# Autodesk Inventor assembly: GFRP_T2_01
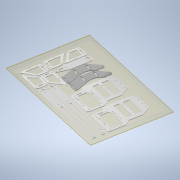
[picture p0: Inventor's stored thumbnail of the model, 180x180]
Saved by Autodesk Inventor 2020 (Build 240168000, 168)
## iProperties
Created: 2021-08-27
Part Number: GFRP_T2_01
Document SubType Name: Assembly
Designer: Masato
Author: Masato
## Documents named in this file (7)
- C:\Users\naoki\Documents\Inventor\CitBrains\git_clone\OpenPlatform167\CAMの確認用\OpenPlatform_ver3_0\cam\GFRP_T2_01.iam
- C:\Users\naoki\Documents\Inventor\CitBrains\git_clone\OpenPlatform167\CAMの確認用\OpenPlatform_ver3_0\cam\Disposable_Board.ipt
- C:\Users\naoki\Documents\Inventor\CitBrains\git_clone\OpenPlatform167\CAMの確認用\OpenPlatform_ver3_0\UpperBody\Head\Head_side_frame.ipt
- C:\Users\naoki\Documents\Inventor\CitBrains\git_clone\OpenPlatform167\CAMの確認用\OpenPlatform_ver3_0\UpperBody\Trunk\Trunk_upper_flank_frame.ipt
- C:\Users\naoki\Documents\Inventor\CitBrains\git_clone\OpenPlatform167\CAMの確認用\OpenPlatform_ver3_0\UpperBody\Arm\ForeArm_outside_frame.ipt
- C:\Users\naoki\Documents\Inventor\CitBrains\git_clone\OpenPlatform167\CAMの確認用\OpenPlatform_ver3_0\UpperBody\Arm\ForeArm_inside_frame.ipt
- C:\Users\naoki\Documents\Inventor\CitBrains\git_clone\OpenPlatform167\CAMの確認用\OpenPlatform_ver3_0\UpperBody\Arm\UpperArm_side_frame.ipt
## Components (13 placed, 6 different names)
1. Disposable_Board:1 — メイト:2, メイト:1, フラッシュ:1, フラッシュ:2, フラッシュ:3, フラッシュ:5, 角度:1, メイト:21, メイト:22, フラッシュ:8
2. ForeArm_inside_frame:1 — メイト:9, メイト:17, メイト:24, メイト:30
3. UpperArm_side_frame:1 — メイト:11, 正接:4, メイト:15, メイト:20, メイト:28, メイト:30
4. UpperArm_side_frame:2 — メイト:17, フラッシュ:7, 正接:5, メイト:25
5. UpperArm_side_frame:3 — フラッシュ:7, 正接:5, メイト:18, メイト:26
6. UpperArm_side_frame:4 — メイト:15, メイト:18, メイト:27, 正接:7
7. UpperArm_side_frame:5 — メイト:20, 正接:6, メイト:29, フラッシュ:8, 正接:7
8. Trunk_upper_flank_frame:1 — フラッシュ:3
9. Trunk_upper_flank_frame:2 — メイト:7, 正接:1, メイト:21
10. ForeArm_outside_frame:2 — メイト:7, フラッシュ:5, 正接:4, メイト:22
11. ForeArm_outside_frame:3 — 正接:6
12. Head_side_frame:1 — 正接:1, 角度:1, メイト:23
13. Head_side_frame:2 — メイト:9, メイト:11
## Component patterns: (2 elements, first: Trunk_upper_flank_frame:1), (2 elements, first: ForeArm_outside_frame:2), (2 elements, first: Head_side_frame:1)
## Relationships (31: Mate 19, Flush 6, Tangent 5, Angle 1)
- メイト:2 [Mate]: Disposable_Board:1
- メイト:1 [Mate]: Disposable_Board:1
- フラッシュ:1 [Flush]: Disposable_Board:1
- フラッシュ:2 [Flush]: Disposable_Board:1
- フラッシュ:3 [Flush] (2 mm): Disposable_Board:1 ↔ Trunk_upper_flank_frame:1
- メイト:7 [Mate] (2.5 mm): Trunk_upper_flank_frame:2 ↔ ForeArm_outside_frame:2
- フラッシュ:5 [Flush] (2 mm): Disposable_Board:1 ↔ ForeArm_outside_frame:2
- 正接:1 [Tangent] (2.5 mm): Trunk_upper_flank_frame:2 ↔ Head_side_frame:1
- 角度:1 [Angle] (90 deg): Disposable_Board:1 ↔ Head_side_frame:1
- メイト:9 [Mate] (2.5 mm): ForeArm_inside_frame:1 ↔ Head_side_frame:2
- メイト:11 [Mate] (2.5 mm): UpperArm_side_frame:1 ↔ Head_side_frame:2
- 正接:4 [Tangent] (2.5 mm): UpperArm_side_frame:1 ↔ ForeArm_outside_frame:2
- メイト:15 [Mate] (2.5 mm): UpperArm_side_frame:1 ↔ UpperArm_side_frame:4
- メイト:17 [Mate] (2.5 mm): ForeArm_inside_frame:1 ↔ UpperArm_side_frame:2
- フラッシュ:7 [Flush]: UpperArm_side_frame:2 ↔ UpperArm_side_frame:3
- 正接:5 [Tangent] (2.5 mm): UpperArm_side_frame:2 ↔ UpperArm_side_frame:3
- メイト:18 [Mate] (2.5 mm): UpperArm_side_frame:3 ↔ UpperArm_side_frame:4
- メイト:20 [Mate] (2.5 mm): UpperArm_side_frame:1 ↔ UpperArm_side_frame:5
- 正接:6 [Tangent] (2.5 mm): UpperArm_side_frame:5 ↔ ForeArm_outside_frame:3
- メイト:21 [Mate]: Disposable_Board:1 ↔ Trunk_upper_flank_frame:2
- メイト:22 [Mate]: Disposable_Board:1 ↔ ForeArm_outside_frame:2
- メイト:23 [Mate]: Head_side_frame:1
- メイト:24 [Mate]: ForeArm_inside_frame:1
- メイト:25 [Mate]: UpperArm_side_frame:2
- メイト:26 [Mate]: UpperArm_side_frame:3
- メイト:27 [Mate]: UpperArm_side_frame:4
- メイト:28 [Mate]: UpperArm_side_frame:1
- メイト:29 [Mate]: UpperArm_side_frame:5
- フラッシュ:8 [Flush] (2 mm): Disposable_Board:1 ↔ UpperArm_side_frame:5
- メイト:30 [Mate] (2.5 mm): ForeArm_inside_frame:1 ↔ UpperArm_side_frame:1
- 正接:7 [Tangent] (2.5 mm): UpperArm_side_frame:4 ↔ UpperArm_side_frame:5
